# Autodesk Inventor assembly: [Face] Dragon
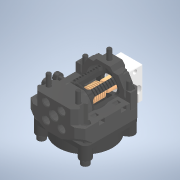
[picture p0: Inventor's stored thumbnail of the model, 180x180]
Saved by Autodesk Inventor 2022 (Build 260153000, 153)
## iProperties
Created: 2021-10-06
Part Number: [Face] Dragon
Document SubType Name: Assembly
Designer: Administrator
Title: [Face] Dragon v4
Author: Administrator
## Documents named in this file (11)
- C:\Users\nicol\Documents\_Origami Printer\Modified EVA Carriage\[Face] Dragon v4.iam
- C:\Users\nicol\Documents\_Origami Printer\Modified EVA Carriage\M3 Hex Nut.ipt
- C:\Users\nicol\Documents\_Origami Printer\Modified EVA Carriage\M3 x 10 mm.ipt
- C:\Users\nicol\Documents\_Origami Printer\Modified EVA Carriage\M3 x 20 mm.ipt
- C:\Users\nicol\Documents\_Origami Printer\Modified EVA Carriage\dragon_face.ipt
- C:\Users\nicol\Documents\_Origami Printer\Modified EVA Carriage\v6_support.ipt
- C:\Users\nicol\Documents\_Origami Printer\Modified EVA Carriage\shroud.ipt
- C:\Users\nicol\Documents\_Origami Printer\Modified EVA Carriage\M3 x 25 mm.ipt
- C:\Users\nicol\Documents\_Origami Printer\Modified EVA Carriage\M3 x 8 mm.ipt
- C:\Users\nicol\Documents\_Origami Printer\Modified EVA Carriage\4010 FAN.ipt
- C:\Users\nicol\Documents\_Origami Printer\Modified EVA Carriage\Dragon _1_.iam
## Components (20 placed, 10 different names)
1. M3  Hex nut :1
2. DIN 912 M3 10 mm:1
3. DIN 912 M3 20 mm:1
4. M3  Hex nut :2
5. dragon_face:1 — Mate:1, Mate:2
6. M3  Hex nut :3
7. DIN 912 M3 20 mm:2
8. v6_support:1
9. shroud:1
10. DIN 912 M3 25 mm:1
11. DIN 912 M3 8 mm:1
12. M3  Hex nut :4
13. 4010 FAN:1
14. DIN 912 M3 25 mm:2 — Mate:2
15. M3  Hex nut :5
16. DIN 912 M3 10 mm:2
17. DIN 912 M3 25 mm:3
18. M3  Hex nut :6
19. Dragon <1>:1 [sub-assembly]
20. DIN 912 M3 25 mm:4 — Mate:1
## Relationships (2: Mate 2)
- Mate:1: dragon_face:1 ↔ DIN 912 M3 25 mm:4
- Mate:2: dragon_face:1 ↔ DIN 912 M3 25 mm:2
